# Autodesk Inventor assembly: RPI and PiTFT
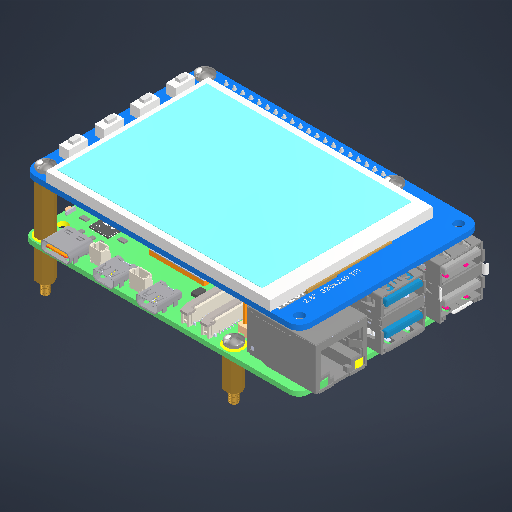
[picture p0: Inventor's stored thumbnail of the model, 512x512]
Saved by Autodesk Inventor 2026 (Build 300175000, 175)
## iProperties
Created: 2025-06-05
Part Number: RPI and PiTFT
Document SubType Name: Assembly
Designer: ckyiu
Author: ckyiu
## Documents named in this file (6)
- C:\Users\ckyiu\Documents\Projects\Chessboard-Design\Design\Core\PCBs\RPI and PiTFT.iam
- C:\Users\ckyiu\Documents\Projects\Chessboard-Design\Design\Core\PCBs\Parts\Raspberry Pi 5.iam
- C:\Users\ckyiu\Documents\Projects\Chessboard-Design\Design\Core\PCBs\Parts\PiTFT 2.8in capacitive.ipt
- C:\Users\ckyiu\Documents\Projects\Chessboard-Design\Design\Hardware\M2.5\Screws\(6mm) 92000A104_Passivated 18-8 Stainless Steel Pan Head Phillips Screws.ipt
- C:\Users\ckyiu\Documents\Projects\Chessboard-Design\Design\Hardware\M2.5\Standoffs\M-F\(16mm) 98952A113_Aluminum Male-Female Threaded Hex Standoff.ipt
- C:\Users\ckyiu\Documents\Projects\Chessboard-Design\Design\Hardware\M2.5\Standoffs\M-F\(10mm) 98952A107_Aluminum Male-Female Threaded Hex Standoff.ipt
## Components (13 placed, 5 different names)
1. Raspberry Pi 5:1 [sub-assembly] — Flush:1, Mate:1, Flush:2, Insert:12, Insert:13, Insert:14, Insert:15, Insert:16, Insert:17, Insert:18, Insert:19
2. PiTFT 2.8in capacitive:1 — Flush:1, Mate:1, Flush:2, Insert:3, Insert:6, Insert:11
3. (6mm) 92000A104_Passivated 18-8 Stainless Steel Pan Head Phillips Screws:1 — Insert:11
4. (6mm) 92000A104_Passivated 18-8 Stainless Steel Pan Head Phillips Screws:2 — Insert:3
5. (6mm) 92000A104_Passivated 18-8 Stainless Steel Pan Head Phillips Screws:3 — Insert:6
6. (6mm) 92000A104_Passivated 18-8 Stainless Steel Pan Head Phillips Screws:4 — Insert:15
7. (16mm) 98952A113_Aluminum Male-Female Threaded Hex Standoff:1 — Insert:12
8. (16mm) 98952A113_Aluminum Male-Female Threaded Hex Standoff:2 — Insert:13
9. (16mm) 98952A113_Aluminum Male-Female Threaded Hex Standoff:3 — Insert:14
10. (10mm) 98952A107_Aluminum Male-Female Threaded Hex Standoff:1 — Insert:16
11. (10mm) 98952A107_Aluminum Male-Female Threaded Hex Standoff:2 — Insert:17
12. (10mm) 98952A107_Aluminum Male-Female Threaded Hex Standoff:3 — Insert:18
13. (10mm) 98952A107_Aluminum Male-Female Threaded Hex Standoff:4 — Insert:19
## Relationships (14: Insert 11, Flush 2, Mate 1)
- Flush:1: Raspberry Pi 5:1 ↔ PiTFT 2.8in capacitive:1
- Mate:1: Raspberry Pi 5:1 ↔ PiTFT 2.8in capacitive:1
- Flush:2: Raspberry Pi 5:1 ↔ PiTFT 2.8in capacitive:1
- Insert:3: PiTFT 2.8in capacitive:1 ↔ (6mm) 92000A104_Passivated 18-8 Stainless Steel Pan Head Phillips Screws:2
- Insert:6: PiTFT 2.8in capacitive:1 ↔ (6mm) 92000A104_Passivated 18-8 Stainless Steel Pan Head Phillips Screws:3
- Insert:11: PiTFT 2.8in capacitive:1 ↔ (6mm) 92000A104_Passivated 18-8 Stainless Steel Pan Head Phillips Screws:1
- Insert:12: Raspberry Pi 5:1 ↔ (16mm) 98952A113_Aluminum Male-Female Threaded Hex Standoff:1
- Insert:13: Raspberry Pi 5:1 ↔ (16mm) 98952A113_Aluminum Male-Female Threaded Hex Standoff:2
- Insert:14: Raspberry Pi 5:1 ↔ (16mm) 98952A113_Aluminum Male-Female Threaded Hex Standoff:3
- Insert:15: Raspberry Pi 5:1 ↔ (6mm) 92000A104_Passivated 18-8 Stainless Steel Pan Head Phillips Screws:4
- Insert:16: Raspberry Pi 5:1 ↔ (10mm) 98952A107_Aluminum Male-Female Threaded Hex Standoff:1
- Insert:17: Raspberry Pi 5:1 ↔ (10mm) 98952A107_Aluminum Male-Female Threaded Hex Standoff:2
- Insert:18: Raspberry Pi 5:1 ↔ (10mm) 98952A107_Aluminum Male-Female Threaded Hex Standoff:3
- Insert:19: Raspberry Pi 5:1 ↔ (10mm) 98952A107_Aluminum Male-Female Threaded Hex Standoff:4
